# Autodesk Inventor assembly: F-wing
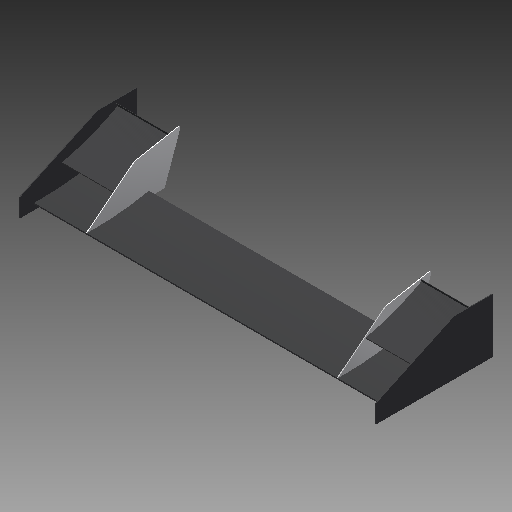
[picture p0: Inventor's stored thumbnail of the model, 512x512]
Saved by Autodesk Inventor 2018 (Build 220112000, 112)
## iProperties
Created: 2017-10-25
Part Number: F-wing
Material: 一般
Document SubType Name: Assembly
Designer: kuwano
Author: kuwano
## Documents named in this file (5)
- Z:\個人フォルダ\kuwano\Inventor\KS-15_Aero_CAD\type5\F-wing\F-wing.iam
- Z:\個人フォルダ\kuwano\Inventor\KS-15_Aero_CAD\type5\F-wing\parts\base\base_booled.ipt
- Z:\個人フォルダ\kuwano\Inventor\KS-15_Aero_CAD\type5\F-wing\parts\stay_middle.ipt
- Z:\個人フォルダ\kuwano\Inventor\KS-15_Aero_CAD\type5\F-wing\parts\side.ipt
- Z:\個人フォルダ\kuwano\Inventor\KS-15_Aero_CAD\type5\F-wing\parts\element_gurnee.ipt
## Components (7 placed, 4 different names)
1. base_booled:1 — フラッシュ:1, フラッシュ:2, フラッシュ:3, メイト:1, メイト:2, メイト:3, メイト:4, メイト:5, メイト:6, メイト:7, メイト:8, フラッシュ:4, フラッシュ:5, フラッシュ:6, フラッシュ:7
2. stay_middle:1 — メイト:1, メイト:4, メイト:6, メイト:13
3. stay_middle:2 — メイト:2, メイト:3, メイト:5, メイト:12
4. side:1 — メイト:8, フラッシュ:4, フラッシュ:7
5. side:2 — メイト:7, フラッシュ:5, フラッシュ:6
6. element_gurnee:1 — メイト:12, メイト:14, フラッシュ:8
7. element_gurnee:2 — メイト:13, メイト:14, フラッシュ:8
## Relationships (19: Mate 11, Flush 8)
- フラッシュ:1 [Flush]: base_booled:1
- フラッシュ:2 [Flush]: base_booled:1
- フラッシュ:3 [Flush]: base_booled:1
- メイト:1 [Mate]: base_booled:1 ↔ stay_middle:1
- メイト:2 [Mate]: base_booled:1 ↔ stay_middle:2
- メイト:3 [Mate]: base_booled:1 ↔ stay_middle:2
- メイト:4 [Mate]: base_booled:1 ↔ stay_middle:1
- メイト:5 [Mate]: base_booled:1 ↔ stay_middle:2
- メイト:6 [Mate]: base_booled:1 ↔ stay_middle:1
- メイト:7 [Mate]: base_booled:1 ↔ side:2
- メイト:8 [Mate]: base_booled:1 ↔ side:1
- フラッシュ:4 [Flush] (20 mm): base_booled:1 ↔ side:1
- フラッシュ:5 [Flush] (20 mm): base_booled:1 ↔ side:2
- フラッシュ:6 [Flush] (55 mm): base_booled:1 ↔ side:2
- フラッシュ:7 [Flush] (55 mm): base_booled:1 ↔ side:1
- メイト:12 [Mate]: stay_middle:2 ↔ element_gurnee:1
- メイト:13 [Mate]: stay_middle:1 ↔ element_gurnee:2
- メイト:14 [Mate]: element_gurnee:1 ↔ element_gurnee:2
- フラッシュ:8 [Flush]: element_gurnee:1 ↔ element_gurnee:2
